# Autodesk Inventor assembly: 3A.03.JS.Wing test assembly
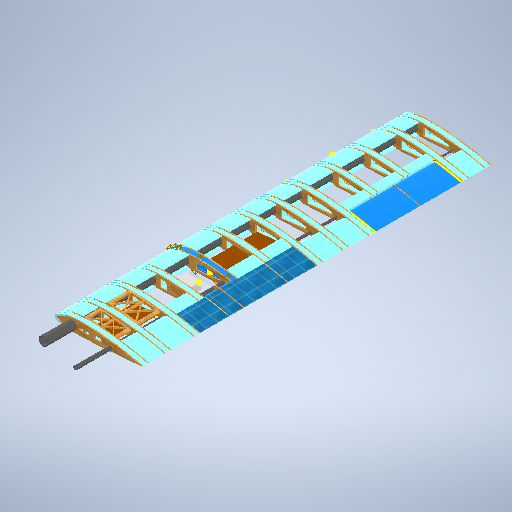
[picture p0: Inventor's stored thumbnail of the model, 512x512]
Saved by Autodesk Inventor 2025.1 (Build 291241000, 241)
## iProperties
Created: 2025-01-14
Part Number: 3A.03.JS.Wing test assembly
Document SubType Name: Assembly
Designer: johan
Author: johan
## Documents named in this file (37)
- C:\Users\johan\OneDrive - University of Bristol\AVDASI\full assembly\S Wing\0)Full Assembly\3A.03.JS.Final Wing Assembly.iam
- C:\Users\johan\OneDrive - University of Bristol\AVDASI\full assembly\S Wing\0)Full Assembly\3A.01.13.JS.Rib 13.iam
- C:\Users\johan\OneDrive - University of Bristol\AVDASI\full assembly\S Wing\0)Full Assembly\3A.04.01.JS.54mm root.iam
- C:\Users\johan\OneDrive - University of Bristol\AVDASI\full assembly\S Wing\0)Full Assembly\3A.01.12.JS.Rib 12.iam
- C:\Users\johan\OneDrive - University of Bristol\AVDASI\full assembly\S Wing\0)Full Assembly\3A.04.02.JS.77mm.iam
- C:\Users\johan\OneDrive - University of Bristol\AVDASI\full assembly\S Wing\0)Full Assembly\3A.01.11.JS.Rib 11.iam
- C:\Users\johan\OneDrive - University of Bristol\AVDASI\full assembly\S Wing\0)Full Assembly\3A.04.03.JS.74.75mm.iam
- C:\Users\johan\OneDrive - University of Bristol\AVDASI\full assembly\S Wing\0)Full Assembly\3A.04.04.90.75mm.iam
- C:\Users\johan\OneDrive - University of Bristol\AVDASI\full assembly\S Wing\0)Full Assembly\3A.01.09.JS.Rib 9.iam
- C:\Users\johan\OneDrive - University of Bristol\AVDASI\full assembly\S Wing\0)Full Assembly\3A.01.08.JS.Rib 8.iam
- C:\Users\johan\OneDrive - University of Bristol\AVDASI\full assembly\S Wing\0)Full Assembly\3A.01.07.JS.Rib 7.iam
- C:\Users\johan\OneDrive - University of Bristol\AVDASI\full assembly\S Wing\0)Full Assembly\3A.04.05.JS.65.5mm.iam
- C:\Users\johan\OneDrive - University of Bristol\AVDASI\full assembly\S Wing\0)Full Assembly\3A.01.06.JS.Rib 6.iam
- C:\Users\johan\OneDrive - University of Bristol\AVDASI\full assembly\S Wing\0)Full Assembly\3A.01.05.JS.Rib 5.iam
- C:\Users\johan\OneDrive - University of Bristol\AVDASI\full assembly\S Wing\0)Full Assembly\3A.04.06.JS.84mm.iam
- C:\Users\johan\OneDrive - University of Bristol\AVDASI\full assembly\S Wing\0)Full Assembly\3A.01.04.JS.Rib 4.iam
- C:\Users\johan\OneDrive - University of Bristol\AVDASI\full assembly\S Wing\0)Full Assembly\3A.01.03.JS.Rib 3.iam
- C:\Users\johan\OneDrive - University of Bristol\AVDASI\full assembly\S Wing\0)Full Assembly\3A.01.02.JS.Rib 2.iam
- C:\Users\johan\OneDrive - University of Bristol\AVDASI\full assembly\S Wing\0)Full Assembly\3A.04.07.JS.54mm tip.iam
- C:\Users\johan\OneDrive - University of Bristol\AVDASI\full assembly\S Wing\0)Full Assembly\3A.01.01.JS.Rib 1.iam
- C:\Users\johan\OneDrive - University of Bristol\AVDASI\full assembly\S Wing\0)Full Assembly\3P.05.07.JS.flap trailing edge 90.ipt
- C:\Users\johan\OneDrive - University of Bristol\AVDASI\full assembly\S Wing\0)Full Assembly\3P.05.01.JS.trailing edge 54mm.ipt
- C:\Users\johan\OneDrive - University of Bristol\AVDASI\full assembly\S Wing\0)Full Assembly\3P.05.04JS.aileron trailing edge.ipt
- C:\Users\johan\OneDrive - University of Bristol\AVDASI\full assembly\S Wing\0)Full Assembly\3P.05.06.JS.flap trailing edge 74.ipt
- C:\Users\johan\OneDrive - University of Bristol\AVDASI\full assembly\S Wing\0)Full Assembly\3P.05.08.JS.trailing edge 65.5mm aileron.ipt
- C:\Users\johan\OneDrive - University of Bristol\AVDASI\full assembly\S Wing\0)Full Assembly\3P.05.09.JS.trailing edge 54mm aileron.ipt
- C:\Users\johan\OneDrive - University of Bristol\AVDASI\full assembly\S Wing\0)Full Assembly\3P.01.GC.MAIN WING SPAR FINAL VERSION - updated.ipt
- C:\Users\johan\OneDrive - University of Bristol\AVDASI\full assembly\S Wing\0)Full Assembly\3P.05.02.JS.trailing edge 77mm.ipt
- C:\Users\johan\OneDrive - University of Bristol\AVDASI\full assembly\S Wing\0)Full Assembly\3A.01.10.JS.Rib 10.iam
- C:\Users\johan\OneDrive - University of Bristol\AVDASI\full assembly\S Wing\0)Full Assembly\access panel test plastic 54.ipt
- C:\Users\johan\OneDrive - University of Bristol\AVDASI\full assembly\S Wing\0)Full Assembly\access panel test plastic 77.ipt
- C:\Users\johan\OneDrive - University of Bristol\AVDASI\full assembly\S Wing\0)Full Assembly\4A.01.02.06-BC-v1-Final Aileron Assembly 80deg.iam
- C:\Users\johan\OneDrive - University of Bristol\AVDASI\full assembly\S Wing\0)Full Assembly\4A.01.01.04-BC-v1-Final Flap v2 Assembly.iam
- C:\Users\johan\OneDrive - University of Bristol\AVDASI\full assembly\S Wing\0)Full Assembly\Plywood Board 11-13.ipt
- C:\Users\johan\OneDrive - University of Bristol\AVDASI\full assembly\S Wing\0)Full Assembly\Plywood Board 7-9.ipt
- C:\Users\johan\OneDrive - University of Bristol\AVDASI\full assembly\S Wing\0)Full Assembly\3P.03.GC.Rear Wing Spar (tapered hollow).ipt
- C:\Users\johan\OneDrive - University of Bristol\AVDASI\full assembly\S Wing\0)Full Assembly\servo mount assembly.iam
## Components (45 placed, 36 different names)
1. 3A.01.01.JS.Rib 1:1 [sub-assembly] — Rigid:24, Rigid:38, Rotational:1, Rotational:7
2. 3A.01.02.JS.Rib 2:1 [sub-assembly] — Rigid:22, Rigid:23
3. 3A.01.03.JS.Rib 3:1 [sub-assembly] — Rigid:20, Rigid:21, Rigid:34
4. 3A.01.04.JS.Rib 4:1 [sub-assembly] — Rigid:18, Rigid:19, Rigid:32, Rigid:33
5. 3A.01.05.JS.Rib 5:1 [sub-assembly] — Rigid:16, Rigid:17, Rotational:6, Mate:1
6. 3A.01.06.JS.Rib 6:1 [sub-assembly] — Rigid:14, Rigid:15, Rigid:37
7. 3A.01.07.JS.Rib 7:1 [sub-assembly] — Rigid:12, Rigid:13, Rigid:40, Mate:6
8. 3A.01.08.JS.Rib 8:1 [sub-assembly] — Rigid:10, Rigid:11, Rigid:31
9. 3A.01.09.JS.Rib 9:1 [sub-assembly] — Rigid:8, Rigid:9, Rigid:29, Mate:5
10. 3A.01.11.JS.Rib 11:1 [sub-assembly] — Rigid:4, Rigid:5, Rotational:4, Mate:3, Mate:4
11. 3A.01.12.JS.Rib 12:1 [sub-assembly] — Rigid:2, Rigid:3, Rigid:39, Mate:7
12. 3A.01.13.JS.Rib 13:1 [sub-assembly] — Rigid:26, Rigid:27, Rigid:44, Rotational:3, Mate:2, Mate:8
13. 3A.04.01.JS.54mm root:1 [sub-assembly] — Rigid:2, Rigid:27, Rigid:44
14. 3A.04.02.JS.77mm:1 [sub-assembly] — Rigid:3, Rigid:4
15. 3A.04.03.JS.74.75mm:1 [sub-assembly] — Rigid:5, Rigid:42
16. 3A.04.04.90.75mm:1 [sub-assembly] — Rigid:8, Rigid:41
17. 3A.04.05.JS.65.5mm:1 [sub-assembly] — Rigid:13, Rigid:14
18. 3A.04.06.JS.84mm:1 [sub-assembly] — Rigid:17, Rigid:18
19. 3A.04.07.JS.54mm tip:1 [sub-assembly] — Rigid:23, Rigid:24
20. 3A.04.04.90.75mm:2 [sub-assembly] — Rigid:9, Rigid:10
21. 3A.04.03.JS.74.75mm:2 [sub-assembly] — Rigid:11, Rigid:12
22. 3A.04.05.JS.65.5mm:2 [sub-assembly] — Rigid:15, Rigid:16
23. 3A.04.06.JS.84mm:2 [sub-assembly] — Rigid:19, Rigid:20
24. 3A.04.06.JS.84mm:3 [sub-assembly] — Rigid:21, Rigid:22
25. 3P.05.01.JS.trailing edge 54mm:1 — Rigid:26
26. 3P.05.04JS.aileron trailing edge:1 — Rigid:32
27. 3P.05.06.JS.flap trailing edge 74:1 — Rigid:31
28. 3P.05.07.JS.flap trailing edge 90:2 — Rigid:29
29. 3P.05.06.JS.flap trailing edge 74:2 — Rigid:45
30. 3P.05.04JS.aileron trailing edge:2 — Rigid:34
31. 3P.05.04JS.aileron trailing edge:3 — Rigid:33
32. 3P.05.08.JS.trailing edge 65.5mm aileron:1 — Rigid:37
33. 3P.05.09.JS.trailing edge 54mm aileron:1 — Rigid:38
34. 3P.01.GC.MAIN WING SPAR FINAL VERSION - updated:1 — Rotational:1
35. 3P.05.02.JS.trailing edge 77mm:1 — Rigid:39, Tangent:1
36. 3P.05.08.JS.trailing edge 65.5mm aileron:2 — Rigid:40
37. 3A.01.10.JS.Rib 10:1 [sub-assembly] — Rigid:41, Rigid:42, Rigid:45, Rotational:5, Rotational:8
38. access panel test plastic 54:1 — Rotational:3, Insert:1, Insert:2, Flush:1, Mate:8
39. access panel test plastic 77:1 — Rotational:4, Insert:1, Insert:2, Flush:1, Mate:7, Tangent:1
40. 4A.01.02.06-BC-v1-Final Aileron Assembly 80deg:1 [sub-assembly] — Rotational:6, Mate:1
41. 4A.01.01.04-BC-v1-Final Flap v2 Assembly:1 [sub-assembly] — Rotational:5
42. Plywood Board 11-13:1 — Mate:2, Mate:3, Mate:4
43. Plywood Board 7-9:1 — Mate:5, Mate:6
44. Rear Wing Spar (tapered hollow):1 — Rotational:7
45. servo mount assembly:1 [sub-assembly] — Rotational:8
## Relationships (55: WeldJoint 36, Mate 8, RevoluteJoint 7, Insert 2, Flush 1, Tangent 1)
- Rigid:2 [WeldJoint]: 3A.01.12.JS.Rib 12:1 ↔ 3A.04.01.JS.54mm root:1
- Rigid:3 [WeldJoint]: 3A.01.12.JS.Rib 12:1 ↔ 3A.04.02.JS.77mm:1
- Rigid:4 [WeldJoint]: 3A.01.11.JS.Rib 11:1 ↔ 3A.04.02.JS.77mm:1
- Rigid:5 [WeldJoint]: 3A.01.11.JS.Rib 11:1 ↔ 3A.04.03.JS.74.75mm:1
- Rigid:8 [WeldJoint]: 3A.01.09.JS.Rib 9:1 ↔ 3A.04.04.90.75mm:1
- Rigid:9 [WeldJoint]: 3A.01.09.JS.Rib 9:1 ↔ 3A.04.04.90.75mm:2
- Rigid:10 [WeldJoint]: 3A.01.08.JS.Rib 8:1 ↔ 3A.04.04.90.75mm:2
- Rigid:11 [WeldJoint]: 3A.01.08.JS.Rib 8:1 ↔ 3A.04.03.JS.74.75mm:2
- Rigid:12 [WeldJoint]: 3A.01.07.JS.Rib 7:1 ↔ 3A.04.03.JS.74.75mm:2
- Rigid:13 [WeldJoint]: 3A.01.07.JS.Rib 7:1 ↔ 3A.04.05.JS.65.5mm:1
- Rigid:14 [WeldJoint]: 3A.01.06.JS.Rib 6:1 ↔ 3A.04.05.JS.65.5mm:1
- Rigid:15 [WeldJoint]: 3A.01.06.JS.Rib 6:1 ↔ 3A.04.05.JS.65.5mm:2
- Rigid:16 [WeldJoint]: 3A.01.05.JS.Rib 5:1 ↔ 3A.04.05.JS.65.5mm:2
- Rigid:17 [WeldJoint]: 3A.01.05.JS.Rib 5:1 ↔ 3A.04.06.JS.84mm:1
- Rigid:18 [WeldJoint]: 3A.01.04.JS.Rib 4:1 ↔ 3A.04.06.JS.84mm:1
- Rigid:19 [WeldJoint]: 3A.01.04.JS.Rib 4:1 ↔ 3A.04.06.JS.84mm:2
- Rigid:20 [WeldJoint]: 3A.01.03.JS.Rib 3:1 ↔ 3A.04.06.JS.84mm:2
- Rigid:21 [WeldJoint]: 3A.01.03.JS.Rib 3:1 ↔ 3A.04.06.JS.84mm:3
- Rigid:22 [WeldJoint]: 3A.01.02.JS.Rib 2:1 ↔ 3A.04.06.JS.84mm:3
- Rigid:23 [WeldJoint]: 3A.01.02.JS.Rib 2:1 ↔ 3A.04.07.JS.54mm tip:1
- Rigid:24 [WeldJoint]: 3A.01.01.JS.Rib 1:1 ↔ 3A.04.07.JS.54mm tip:1
- Rigid:26 [WeldJoint]: 3A.01.13.JS.Rib 13:1 ↔ 3P.05.01.JS.trailing edge 54mm:1
- Rigid:27 [WeldJoint]: 3A.01.13.JS.Rib 13:1 ↔ 3A.04.01.JS.54mm root:1
- Rigid:29 [WeldJoint]: 3A.01.09.JS.Rib 9:1 ↔ 3P.05.07.JS.flap trailing edge 90:2
- Rigid:31 [WeldJoint]: 3A.01.08.JS.Rib 8:1 ↔ 3P.05.06.JS.flap trailing edge 74:1
- Rigid:32 [WeldJoint]: 3A.01.04.JS.Rib 4:1 ↔ 3P.05.04JS.aileron trailing edge:1
- Rigid:33 [WeldJoint]: 3A.01.04.JS.Rib 4:1 ↔ 3P.05.04JS.aileron trailing edge:3
- Rigid:34 [WeldJoint]: 3A.01.03.JS.Rib 3:1 ↔ 3P.05.04JS.aileron trailing edge:2
- Rigid:37 [WeldJoint]: 3A.01.06.JS.Rib 6:1 ↔ 3P.05.08.JS.trailing edge 65.5mm aileron:1
- Rigid:38 [WeldJoint]: 3A.01.01.JS.Rib 1:1 ↔ 3P.05.09.JS.trailing edge 54mm aileron:1
- Rigid:39 [WeldJoint]: 3A.01.12.JS.Rib 12:1 ↔ 3P.05.02.JS.trailing edge 77mm:1
- Rigid:40 [WeldJoint]: 3A.01.07.JS.Rib 7:1 ↔ 3P.05.08.JS.trailing edge 65.5mm aileron:2
- Rigid:41 [WeldJoint]: 3A.04.04.90.75mm:1 ↔ 3A.01.10.JS.Rib 10:1
- Rigid:42 [WeldJoint]: 3A.04.03.JS.74.75mm:1 ↔ 3A.01.10.JS.Rib 10:1
- Rigid:44 [WeldJoint]: 3A.01.13.JS.Rib 13:1 ↔ 3A.04.01.JS.54mm root:1
- Rigid:45 [WeldJoint]: 3P.05.06.JS.flap trailing edge 74:2 ↔ 3A.01.10.JS.Rib 10:1
- Rotational:1 [RevoluteJoint]: 3A.01.01.JS.Rib 1:1 ↔ 3P.01.GC.MAIN WING SPAR FINAL VERSION - updated:1
- Rotational:3 [RevoluteJoint]: 3A.01.13.JS.Rib 13:1 ↔ access panel test plastic 54:1
- Rotational:4 [RevoluteJoint]: 3A.01.11.JS.Rib 11:1 ↔ access panel test plastic 77:1
- Rotational:5 [RevoluteJoint]: 3A.01.10.JS.Rib 10:1 ↔ 4A.01.01.04-BC-v1-Final Flap v2 Assembly:1
- Rotational:6 [RevoluteJoint]: 3A.01.05.JS.Rib 5:1 ↔ 4A.01.02.06-BC-v1-Final Aileron Assembly 80deg:1
- Mate:1: 3A.01.05.JS.Rib 5:1 ↔ 4A.01.02.06-BC-v1-Final Aileron Assembly 80deg:1
- Mate:2: 3A.01.13.JS.Rib 13:1 ↔ Plywood Board 11-13:1
- Mate:3: 3A.01.11.JS.Rib 11:1 ↔ Plywood Board 11-13:1
- Mate:4: 3A.01.11.JS.Rib 11:1 ↔ Plywood Board 11-13:1
- Mate:5: 3A.01.09.JS.Rib 9:1 ↔ Plywood Board 7-9:1
- Mate:6: 3A.01.07.JS.Rib 7:1 ↔ Plywood Board 7-9:1
- Insert:1 (23 mm): access panel test plastic 54:1 ↔ access panel test plastic 77:1
- Insert:2 (23 mm): access panel test plastic 54:1 ↔ access panel test plastic 77:1
- Flush:1: access panel test plastic 54:1 ↔ access panel test plastic 77:1
- Mate:7: 3A.01.12.JS.Rib 12:1 ↔ access panel test plastic 77:1
- Mate:8: 3A.01.13.JS.Rib 13:1 ↔ access panel test plastic 54:1
- Tangent:1 (11 mm): 3P.05.02.JS.trailing edge 77mm:1 ↔ access panel test plastic 77:1
- Rotational:7 [RevoluteJoint]: 3A.01.01.JS.Rib 1:1 ↔ Rear Wing Spar (tapered hollow):1
- Rotational:8 [RevoluteJoint]: 3A.01.10.JS.Rib 10:1 ↔ servo mount assembly:1
